# Autodesk Inventor assembly: EsagonoScreeenChiuso
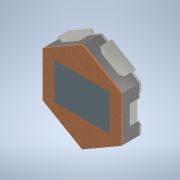
[picture p0: Inventor's stored thumbnail of the model, 180x180]
Saved by Autodesk Inventor 2020 (Build 240168000, 168)
## iProperties
Created: 2020-04-22
Part Number: EsagonoScreeenChiuso
Document SubType Name: Assembly
Designer: Samuele
Author: Samuele
## Documents named in this file (5)
- C:\EsagoniMalsani\ModelliComponenti\EsagonoScreeenChiuso.iam
- C:\EsagoniMalsani\ModelliComponenti\HexagoneBack.ipt
- C:\EsagoniMalsani\ModelliComponenti\Componenti\TouchLCD.ipt
- C:\EsagoniMalsani\ModelliComponenti\Esagoni\FrontalinoWood.ipt
- C:\EsagoniMalsani\ModelliComponenti\Esagoni\HexagoneScreen.ipt
## Components (4 placed, 4 different names)
1. HexagoneScreen:1 — Flush:1, Mate:1, Flush:2, Mate:4, Mate:5, Mate:6
2. TouchLCD:1 — Mate:2, Mate:3, Flush:3
3. HexagoneBack:1 — Mate:4, Mate:5, Mate:6
4. FrontalinoWood:1 — Flush:1, Mate:1, Flush:2, Mate:2, Mate:3, Flush:3
## Relationships (9: Mate 6, Flush 3)
- Flush:1: HexagoneScreen:1 ↔ FrontalinoWood:1
- Mate:1: HexagoneScreen:1 ↔ FrontalinoWood:1
- Flush:2: HexagoneScreen:1 ↔ FrontalinoWood:1
- Mate:2: TouchLCD:1 ↔ FrontalinoWood:1
- Mate:3: TouchLCD:1 ↔ FrontalinoWood:1
- Flush:3: TouchLCD:1 ↔ FrontalinoWood:1
- Mate:4: HexagoneScreen:1 ↔ HexagoneBack:1
- Mate:5: HexagoneScreen:1 ↔ HexagoneBack:1
- Mate:6: HexagoneScreen:1 ↔ HexagoneBack:1
